# Autodesk Inventor assembly: Assy_wrist_fore
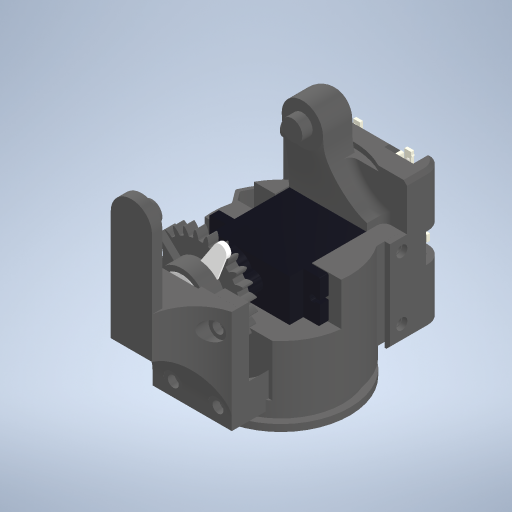
[picture p0: Inventor's stored thumbnail of the model, 512x512]
Saved by Autodesk Inventor 2024.1 (Build 281209000, 209)
## iProperties
Created: 2025-03-02
Part Number: Assy_wrist_fore
Document SubType Name: Assembly
Designer: hibik
Author: hibik
## Documents named in this file (9)
- C:\Users\hibik\Documents\Robomech\RESCUE\ORCA\hard\arm\Assy_wrist_fore.iam
- C:\Users\hibik\Documents\Robomech\RESCUE\ORCA\hard\arm\wrist_wrist.ipt
- C:\Users\hibik\Documents\Robomech\RESCUE\ORCA\hard\std_parts\Miusei_ms18.ipt
- C:\Users\hibik\Documents\Robomech\RESCUE\ORCA\hard\arm\hand_gear_wrist.ipt
- C:\Users\hibik\Documents\Robomech\RESCUE\ORCA\hard\std_parts\Miusei_hone_short.ipt
- C:\Users\hibik\Documents\Robomech\RESCUE\ORCA\hard\arm\wrist_hand_connector.ipt
- C:\Users\hibik\Documents\Robomech\RESCUE\ORCA\hard\std_parts\bearing_6_10_3.ipt
- C:\Users\hibik\Documents\Robomech\RESCUE\ORCA\hard\board\CORE_model\md.iam
- C:\Users\hibik\Documents\Robomech\RESCUE\ORCA\hard\arm\wrist_board_cover.ipt
## Components (8 placed, 8 different names)
1. Miusei_ms18:1 — 挿入:1, メイト:7, メイト:8, メイト:9
2. hand_gear_wrist:1 — 挿入:2, 挿入:17
3. Miusei_hone_short:1 — 挿入:1, 挿入:2
4. wrist_hand_connector:1 — 挿入:15, 挿入:16
5. wrist_wrist:1 — 挿入:15, 挿入:16, メイト:7, メイト:8, メイト:9, 挿入:18, 角度:1, フラッシュ:1, フラッシュ:2, メイト:10, フラッシュ:3, フラッシュ:4, フラッシュ:5
6. bearing_6_10_3:2 — 挿入:17
7. md:1 [sub-assembly] — 挿入:18, 角度:1
8. wrist_board_cover:1 — フラッシュ:1, フラッシュ:2, メイト:10
## Relationships (16: Insert 6, Flush 5, Mate 4, Angle 1)
- 挿入:1 [Insert] (2 mm): Miusei_ms18:1 ↔ Miusei_hone_short:1
- 挿入:2 [Insert]: hand_gear_wrist:1 ↔ Miusei_hone_short:1
- 挿入:15 [Insert]: wrist_hand_connector:1 ↔ wrist_wrist:1
- 挿入:16 [Insert]: wrist_hand_connector:1 ↔ wrist_wrist:1
- メイト:7 [Mate]: Miusei_ms18:1 ↔ wrist_wrist:1
- メイト:8 [Mate]: Miusei_ms18:1 ↔ wrist_wrist:1
- メイト:9 [Mate]: Miusei_ms18:1 ↔ wrist_wrist:1
- 挿入:17 [Insert]: hand_gear_wrist:1 ↔ bearing_6_10_3:2
- 挿入:18 [Insert]: wrist_wrist:1 ↔ md:1
- 角度:1 [Angle] (0 deg): wrist_wrist:1 ↔ md:1
- フラッシュ:1 [Flush]: wrist_wrist:1 ↔ wrist_board_cover:1
- フラッシュ:2 [Flush]: wrist_wrist:1 ↔ wrist_board_cover:1
- メイト:10 [Mate] (8 mm): wrist_wrist:1 ↔ wrist_board_cover:1
- フラッシュ:3 [Flush]: wrist_wrist:1
- フラッシュ:4 [Flush] (-6 mm): wrist_wrist:1
- フラッシュ:5 [Flush]: wrist_wrist:1
